# Autodesk Inventor assembly: MainModule
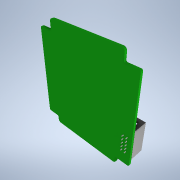
[picture p0: Inventor's stored thumbnail of the model, 180x180]
Saved by Autodesk Inventor 2021 (Build 250183000, 183)
## iProperties
Created: 2021-05-14
Part Number: MainModule
Document SubType Name: Assembly
Designer: ermoz
Author: ermoz
## Documents named in this file (7)
- D:\Moje Wyczyny\My_Poor_Projects\Sneak100_MiniSumo\minisumo-sneak100\mechanics\ElectricElements\MainModule.iam
- D:\Moje Wyczyny\My_Poor_Projects\Sneak100_MiniSumo\minisumo-sneak100\mechanics\ElectricElements\MainBoard.ipt
- D:\Moje Wyczyny\My_Poor_Projects\Sneak100_MiniSumo\minisumo-sneak100\mechanics\PreMadeParts\IDC_10_pin_connector.ipt
- D:\Moje Wyczyny\My_Poor_Projects\Sneak100_MiniSumo\minisumo-sneak100\mechanics\PreMadeParts\TSOP4838.ipt
- D:\Moje Wyczyny\My_Poor_Projects\Sneak100_MiniSumo\minisumo-sneak100\mechanics\PreMadeParts\STM32F303RE_LQFP64.ipt
- D:\Moje Wyczyny\My_Poor_Projects\Sneak100_MiniSumo\minisumo-sneak100\mechanics\PreMadeParts\SSD1306.ipt
- D:\Moje Wyczyny\My_Poor_Projects\Sneak100_MiniSumo\minisumo-sneak100\mechanics\PreMadeParts\TactSwitch_6x6_8mm_SMD.ipt
## Components (8 placed, 6 different names)
1. MainBoard:1 — Mate:1, Mate:3, Mate:7, Flush:1, Mate:8, Mate:9, Angle:1, Mate:17, Mate:18, Mate:19
2. IDC_10_pin_connector:1 — Mate:1, Flush:1
3. STM32F303RE_LQFP64:1 — Mate:3
4. TSOP4838:5 — Mate:7
5. SSD1306:1 — Mate:8, Mate:10, Angle:2
6. TactSwitch_6x6_8mm_SMD:1 — Mate:17, Symmetry:1, Flush:2
7. TactSwitch_6x6_8mm_SMD:2 — Mate:18, Mate:20, Angle:3, Flush:2, Flush:3
8. TactSwitch_6x6_8mm_SMD:3 — Mate:19, Symmetry:1, Flush:3
## Relationships (20: Mate 13, Flush 3, Angle 3, Symmetry 1)
- Mate:1: MainBoard:1 ↔ IDC_10_pin_connector:1
- Mate:3: MainBoard:1 ↔ STM32F303RE_LQFP64:1
- Mate:7 (3 mm): MainBoard:1 ↔ TSOP4838:5
- Flush:1: MainBoard:1 ↔ IDC_10_pin_connector:1
- Mate:8 (4 mm): MainBoard:1 ↔ SSD1306:1
- Mate:9: MainBoard:1
- Angle:1 (0 deg): MainBoard:1
- Mate:10: SSD1306:1
- Angle:2 (0 deg): SSD1306:1
- Mate:11
- Mate:16
- Mate:17: MainBoard:1 ↔ TactSwitch_6x6_8mm_SMD:1
- Mate:18: MainBoard:1 ↔ TactSwitch_6x6_8mm_SMD:2
- Mate:19: MainBoard:1 ↔ TactSwitch_6x6_8mm_SMD:3
- Mate:20: TactSwitch_6x6_8mm_SMD:2
- Angle:3 (0 deg): TactSwitch_6x6_8mm_SMD:2
- Symmetry:1: TactSwitch_6x6_8mm_SMD:1 ↔ TactSwitch_6x6_8mm_SMD:3
- Mate:21
- Flush:2: TactSwitch_6x6_8mm_SMD:1 ↔ TactSwitch_6x6_8mm_SMD:2
- Flush:3: TactSwitch_6x6_8mm_SMD:2 ↔ TactSwitch_6x6_8mm_SMD:3
